# Autodesk Inventor assembly: POM_T5_06
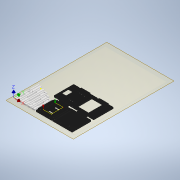
[picture p0: Inventor's stored thumbnail of the model, 180x180]
Saved by Autodesk Inventor 2020 (Build 240168000, 168)
## iProperties
Created: 2021-08-27
Part Number: POM_T5_06
Document SubType Name: Assembly
Designer: Masato
Author: Masato
## Documents named in this file (11)
- C:\Users\naoki\Documents\Inventor\CitBrains\git_clone\OpenPlatform4_0\jig\OpenPlatform_ver3_0\cam\POM_T5_06.iam
- C:\Users\naoki\Documents\Inventor\CitBrains\git_clone\OpenPlatform4_0\jig\OpenPlatform_ver3_0\cam\Disposable_Board.ipt
- C:\Users\naoki\Documents\Inventor\CitBrains\git_clone\OpenPlatform4_0\jig\OpenPlatform_ver3_0\JIG\Cockpit_lower_front_frame_jig.ipt
- C:\Users\naoki\Documents\Inventor\CitBrains\git_clone\OpenPlatform4_0\jig\OpenPlatform_ver3_0\JIG\Cockpit_lower_side_frame_jig_01.ipt
- C:\Users\naoki\Documents\Inventor\CitBrains\git_clone\OpenPlatform4_0\jig\OpenPlatform_ver3_0\JIG\Cockpit_lower_side_frame_jig_02.ipt
- C:\Users\naoki\Documents\Inventor\CitBrains\git_clone\OpenPlatform4_0\jig\OpenPlatform_ver3_0\JIG\Cockpit_upper_bottom_frame_jig.ipt
- C:\Users\naoki\Documents\Inventor\CitBrains\git_clone\OpenPlatform4_0\jig\OpenPlatform_ver3_0\JIG\Cockpit_upper_front_frame_jig.ipt
- C:\Users\naoki\Documents\Inventor\CitBrains\git_clone\OpenPlatform4_0\jig\OpenPlatform_ver3_0\JIG\Cockpit_upper_side_frame_jig.ipt
- C:\Users\naoki\Documents\Inventor\CitBrains\git_clone\OpenPlatform4_0\jig\OpenPlatform_ver3_0\UpperBody\Head\Camera_root_frame.ipt
- C:\Users\naoki\Documents\Inventor\CitBrains\git_clone\OpenPlatform4_0\jig\OpenPlatform_ver3_0\UpperBody\Cockpit\Cockpit_upper_back_door.ipt
- C:\Users\naoki\Documents\Inventor\CitBrains\git_clone\OpenPlatform4_0\jig\OpenPlatform_ver3_0\UpperBody\Cockpit\Cockpit_upper_bottom_frame.ipt
## Components (10 placed, 10 different names)
1. Disposable_Board:1 — メイト:2, メイト:1, フラッシュ:1, フラッシュ:2, メイト:4, メイト:5, メイト:6, メイト:7, メイト:8, メイト:9, フラッシュ:3, フラッシュ:4, フラッシュ:11
2. Cockpit_lower_front_frame_jig:1 — メイト:4, フラッシュ:3, フラッシュ:4, メイト:10, フラッシュ:5, フラッシュ:9, メイト:14
3. Cockpit_lower_side_frame_jig_01:1 — メイト:5, メイト:13, フラッシュ:8, メイト:18
4. Cockpit_lower_side_frame_jig_02:1 — メイト:6, フラッシュ:9, メイト:14
5. Cockpit_upper_bottom_frame_jig:1 — メイト:7, メイト:10, メイト:11, フラッシュ:5, フラッシュ:6
6. Cockpit_upper_front_frame_jig:1 — メイト:8, メイト:11, メイト:12, フラッシュ:6, フラッシュ:7
7. Cockpit_upper_side_frame_jig:1 — メイト:9, メイト:12, メイト:13, フラッシュ:7, フラッシュ:8
8. Camera_root_frame:1 — メイト:15, フラッシュ:10, フラッシュ:11, メイト:18, メイト:19, メイト:20
9. Cockpit_upper_back_door:1 — メイト:16, フラッシュ:10, メイト:19, フラッシュ:12
10. Cockpit_upper_bottom_frame:1 — メイト:17, メイト:20, フラッシュ:12
## Relationships (31: Mate 19, Flush 12)
- メイト:2 [Mate]: Disposable_Board:1
- メイト:1 [Mate]: Disposable_Board:1
- フラッシュ:1 [Flush]: Disposable_Board:1
- フラッシュ:2 [Flush]: Disposable_Board:1
- メイト:4 [Mate]: Disposable_Board:1 ↔ Cockpit_lower_front_frame_jig:1
- メイト:5 [Mate]: Disposable_Board:1 ↔ Cockpit_lower_side_frame_jig_01:1
- メイト:6 [Mate]: Disposable_Board:1 ↔ Cockpit_lower_side_frame_jig_02:1
- メイト:7 [Mate]: Disposable_Board:1 ↔ Cockpit_upper_bottom_frame_jig:1
- メイト:8 [Mate]: Disposable_Board:1 ↔ Cockpit_upper_front_frame_jig:1
- メイト:9 [Mate]: Disposable_Board:1 ↔ Cockpit_upper_side_frame_jig:1
- フラッシュ:3 [Flush] (2 mm): Disposable_Board:1 ↔ Cockpit_lower_front_frame_jig:1
- フラッシュ:4 [Flush] (2 mm): Disposable_Board:1 ↔ Cockpit_lower_front_frame_jig:1
- メイト:10 [Mate] (2.5 mm): Cockpit_lower_front_frame_jig:1 ↔ Cockpit_upper_bottom_frame_jig:1
- メイト:11 [Mate] (2.5 mm): Cockpit_upper_bottom_frame_jig:1 ↔ Cockpit_upper_front_frame_jig:1
- メイト:12 [Mate] (2.5 mm): Cockpit_upper_front_frame_jig:1 ↔ Cockpit_upper_side_frame_jig:1
- メイト:13 [Mate] (2.5 mm): Cockpit_lower_side_frame_jig_01:1 ↔ Cockpit_upper_side_frame_jig:1
- フラッシュ:5 [Flush]: Cockpit_lower_front_frame_jig:1 ↔ Cockpit_upper_bottom_frame_jig:1
- フラッシュ:6 [Flush]: Cockpit_upper_bottom_frame_jig:1 ↔ Cockpit_upper_front_frame_jig:1
- フラッシュ:7 [Flush]: Cockpit_upper_front_frame_jig:1 ↔ Cockpit_upper_side_frame_jig:1
- フラッシュ:8 [Flush]: Cockpit_lower_side_frame_jig_01:1 ↔ Cockpit_upper_side_frame_jig:1
- フラッシュ:9 [Flush]: Cockpit_lower_front_frame_jig:1 ↔ Cockpit_lower_side_frame_jig_02:1
- メイト:14 [Mate] (2.5 mm): Cockpit_lower_front_frame_jig:1 ↔ Cockpit_lower_side_frame_jig_02:1
- メイト:15 [Mate]: Camera_root_frame:1
- メイト:16 [Mate]: Cockpit_upper_back_door:1
- メイト:17 [Mate]: Cockpit_upper_bottom_frame:1
- フラッシュ:10 [Flush]: Camera_root_frame:1 ↔ Cockpit_upper_back_door:1
- フラッシュ:11 [Flush] (-2 mm): Disposable_Board:1 ↔ Camera_root_frame:1
- メイト:18 [Mate] (2.5 mm): Cockpit_lower_side_frame_jig_01:1 ↔ Camera_root_frame:1
- メイト:19 [Mate] (2.5 mm): Camera_root_frame:1 ↔ Cockpit_upper_back_door:1
- メイト:20 [Mate] (2.5 mm): Camera_root_frame:1 ↔ Cockpit_upper_bottom_frame:1
- フラッシュ:12 [Flush]: Cockpit_upper_back_door:1 ↔ Cockpit_upper_bottom_frame:1
